# Autodesk Inventor assembly: MBRAC45-2-10
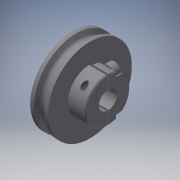
[picture p0: Inventor's stored thumbnail of the model, 180x180]
Saved by Autodesk Inventor 2019 (Build 230136000, 136)
## iProperties
Category: PARTsolutions
Company: MISUMI
Created: 2024-03-05
Part Number: MBRAC45-2-10
Catalog Web Link: www.cadenas.de
Description: MBRC, MBRAC-Pulleys for Round Belts - Clamping
Vendor: MISUMI
Document SubType Name: Assembly
Designer: psAdmin
Manufacturer: MISUMI
Mass: 18.5495 g
Surface Area: 79.8746 cm^2
Volume: 18.5495 cm^3
Density: 1 g/cm^3
Title: MBRAC45-2-10
Author: Cadenas PARTsolutions
Comments: Pulleys for Round Belts - Clamping
PSOL_IDENT_0: {$CADENAS_DATA/23d-libs/misumi/metric/52_belts_pulleys/mbrc_asmtab.prj},190 {VTYP=3D},{STYP=ASSTAB},
PSOL_IDENT_1: {NB=MBRAC45-2-10},{LINA=MBRAC45-2-10},{NN=MBRC, MBRAC},{DATE=30.06.2021 13:25:55},{GEOMDATE=02.09.20
PSOL_IDENT_2: 14},{VERSION=},{LINEID=30},{WBVAR=MAT,PD,DDS},{WBNUMERIC=PD,DDS}  {NB=MBRAC45-2-10},{LINA=MBRAC45-2-
PSOL_IDENT_3: 10},{KT=DUMMY},{PN=MBRAC45-2-10},{TYPE=MBRAC},{MAT=2},{ST=Clear Anodizing},{AC=Hexagon Socket Head C
PSOL_IDENT_4: ap Screw (2Pcs.) Stainless Steel},{PD=45},{PD0=23,28,30,40,45,48,60,80},{R=2.0},{DDS=10.00},{DS0=5,6
PSOL_IDENT_5: ,6.35,8,10,11,12},{D=25},{D1=47},{D2=41},{L=20},{T=10},{LL=4.5},{X=9.0},{Y=4.5},{M=M4},{MM=4},{MMMIN=
PSOL_IDENT_6: 3.242},{DD1=8.0},{DD2=3.5},{PPATH=mbrc_templ.prj}
NB: MBRAC45-2-10
NN: MBRC, MBRAC
NT: Pulleys for Round Belts - Clamping
NBSYN: $PN.
LINA: MBRAC45-2-10
CATALOG: Misumi
PN: MBRAC45-2-10
MAT: A5052
ST: Clear Anodizing
AC: Hexagon Socket Head Cap Screw (2Pcs.) Stainless Steel
PD: 45
R: 2
DDS: 10
D: 25
D1: 47
D2: 41
L: 20
T: 10
LL: 4.5
X: 9
Y: 4.5
M: M4
SUPPLIER: MISUMI
ARTICLENO: MBRAC45-2-10
BOMINFO: MBRAC45-2-10
CREATOR: CADENAS GmbH
## Documents named in this file (4)
- e:\temp\worker_COMMON_2\temp\tmp_2196_120_Z2u6s\format_0\MBRAC45-2-10.iam
- e:\temp\worker_COMMON_2\temp\tmp_2196_120_Z2u6s\format_0\MBRAC45-2-10p1.ipt
- e:\temp\worker_COMMON_2\temp\tmp_2196_120_Z2u6s\format_0\MBRAC45-2-10p2.ipt
- e:\temp\worker_COMMON_2\temp\tmp_2196_120_Z2u6s\format_0\M4x10p3.ipt
## Components (4 placed, 3 different names)
1. MBRAC45-2-10p1:1 — part1_to_part2_XY@1 <-> part2_to_part1_XY@2, part1_to_part2_Z@1 <-> part2_to_part1_Z@2, part1_to_part2_YZ@1 <-> part2_to_part1_YZ@2
2. MBRAC45-2-10p2:1 — part1_to_part2_XY@1 <-> part2_to_part1_XY@2, part1_to_part2_Z@1 <-> part2_to_part1_Z@2, part1_to_part2_YZ@1 <-> part2_to_part1_YZ@2, part2_to_screw1_Z@2 <-> IP1_Z@3, part2_to_screw2_Z@2 <-> IP1_Z@4
3. M4x10p3:1 — part2_to_screw1_Z@2 <-> IP1_Z@3
4. M4x10p3:2 — part2_to_screw2_Z@2 <-> IP1_Z@4
## Relationships (5: Mate 3, Flush 1, Angle 1)
- part1_to_part2_XY@1 <-> part2_to_part1_XY@2 [Flush]: MBRAC45-2-10p1:1 ↔ MBRAC45-2-10p2:1
- part1_to_part2_Z@1 <-> part2_to_part1_Z@2 [Mate]: MBRAC45-2-10p1:1 ↔ MBRAC45-2-10p2:1
- part1_to_part2_YZ@1 <-> part2_to_part1_YZ@2 [Angle] (0 deg): MBRAC45-2-10p1:1 ↔ MBRAC45-2-10p2:1
- part2_to_screw1_Z@2 <-> IP1_Z@3 [Mate]: MBRAC45-2-10p2:1 ↔ M4x10p3:1
- part2_to_screw2_Z@2 <-> IP1_Z@4 [Mate]: MBRAC45-2-10p2:1 ↔ M4x10p3:2
